# Autodesk Inventor assembly: foreArm
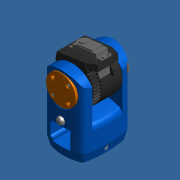
[picture p0: Inventor's stored thumbnail of the model, 180x180]
Saved by Autodesk Inventor 2014 SP2 (Build 180246200, 246)
## iProperties
Created: 2014-12-14
Part Number: foreArm
Document SubType Name: Assembly
Designer: 4ndreas
Mass: 1030.82 g
Surface Area: 1484.59 cm^2
Volume: 608.467 cm^3
Density: 1.69413 g/cm^3
Author: 4ndreas
## Documents named in this file (21)
- C:\Users\4ndreas\Documents\Inventor\RobotARm\foreArm.iam
- C:\Users\4ndreas\Documents\Inventor\RobotARm\RotaryArm.ipt
- C:\Users\4ndreas\Documents\Inventor\RobotARm\foreArm\Konstruktions-Assistent\Stirnräder1.iam
- C:\Users\4ndreas\Documents\Inventor\RobotARm\foreArm\Konstruktions-Assistent\Stirnräder2.iam
- C:\Users\4ndreas\Documents\Inventor\RobotARm\Nema11.ipt
- C:\Users\4ndreas\Documents\Inventor\RobotARm\foreArm\foreArm.ipt
- C:\Users\4ndreas\Documents\Inventor\RobotARm\foreArm\Konstruktions-Assistent\Stirnzahnrad12.ipt
- C:\Users\4ndreas\Documents\Inventor\Content Center Files\R2014\DIN 625 SKF - SKF 618_6_5mm.ipt
- C:\Users\4ndreas\Documents\Inventor\Content Center Files\R2014\de-DE\DIN BEARING(1)\DIN 625 SKF - SKF 626.ipt
- C:\Users\4ndreas\Documents\Inventor\RobotARm\Abdeckung.ipt
- C:\Users\4ndreas\Documents\Inventor\RobotARm\servo.ipt
- C:\Users\4ndreas\Documents\Inventor\Content Center Files\R2014\Leufter_30mm.ipt
- C:\Users\4ndreas\Documents\Inventor\RobotARm\foreArm\Konstruktions-Assistent\Welle1.iam
- C:\Users\4ndreas\Documents\Inventor\RobotARm\6mm Wellen klemme.ipt
- C:\Users\4ndreas\Documents\Inventor\Content Center Files\R2014\de-DE\DIN 913\DIN 913 - M3 x 4.ipt
- C:\Users\4ndreas\Documents\Inventor\Content Center Files\R2014\de-DE\DIN 931-1\DIN 931-1 - M6 x 35.ipt
- C:\Users\4ndreas\Documents\Inventor\Content Center Files\R2014\de-DE\DIN 433-1  A\DIN 433 - 6,4.ipt
- C:\Users\4ndreas\Documents\Inventor\Content Center Files\R2014\de-DE\DIN 985\DIN 985 - M6.ipt
- C:\Users\4ndreas\Documents\Inventor\Content Center Files\R2014\de-DE\DIN 912\DIN 912 - M4 x 0,7 x 25 x 23,25.ipt
- C:\Users\4ndreas\Documents\Inventor\Content Center Files\R2014\de-DE\DIN 934\DIN 934 - M4 x 0,7.ipt
- C:\Users\4ndreas\Documents\Inventor\Content Center Files\R2014\de-DE\DIN EN ISO 7046-2 H\DIN EN ISO 7046-2 H - M3x10 - 8.8 - H1.ipt
## Components (30 placed, 19 different names)
1. RotaryArm:1 — Passend:3, Passend:5, Passend:7, Passend:10, Winkel:1, Fluchtend:1, Passend:15, Passend:17, Passend:22, Passend:23, Passend:24, Passend:25, Passend:26, Passend:27, Passend:28, Fluchtend:2, Passend:29, Passend:30, Winkel:2, Winkel:3, Passend:38, Passend:39, Passend:40, Passend:41, Passend:42, Passend:43, Winkel:4, Fluchtend:4, Passend:53, Passend:54, Passend:59, Passend:60, Fluchtend:5, Passend:64, Passend:65, Winkel:6, Winkel:7, Passend:68, Passend:69, Passend:70
2. Stirnräder:1 [sub-assembly] — Passend:1, Passend:2, Passend:10, Fluchtend:3
3. Stirnräder:2 [sub-assembly] — Passend:13, Passend:14, Passend:15, Passend:16
4. Nema11:1 — Passend:11, Winkel:1, Passend:41
5. foreArm:1 — Passend:17, Passend:18, Drehung:1, Passend:36, Passend:37, Passend:57, Passend:58
6. Stirnzahnrad1:1 — Passend:19, Passend:20, Drehung:1
7. DIN 625 SKF 618/6:1 — Passend:21, Passend:24, Passend:46
8. DIN 625 SKF 618/6:2 — Passend:22, Passend:23
9. DIN 625 SKF 626:1 — Passend:26, Passend:27, Passend:49, Passend:50
10. DIN 625 SKF 626:2 — Passend:25, Passend:28, Passend:47, Passend:48
11. Abdeckung:1 — Passend:29, Passend:30, Passend:31, Passend:32, Passend:66, Passend:67
12. servo:1 — Passend:35, Passend:37, Winkel:3
13. Abdeckung:2 — Passend:38, Passend:39, Passend:40
14. Leufter_30mm:1 — Passend:42, Passend:43, Winkel:4
15. Welle:1 [sub-assembly] — Passend:44, Fluchtend:3, Passend:45
16. 6mm Wellen klemme:1 — Fluchtend:4, Passend:45, Passend:46, Zylindrisch:1
17. DIN 913 M3 x 4:1 — Zylindrisch:1
18. DIN 931-1 - ersetzt durch DIN EN 24014 M6 x 35:1 — Passend:47, Passend:48, Passend:52, Passend:56
19. DIN 931-1 - ersetzt durch DIN EN 24014 M6 x 35:2 — Passend:49, Passend:50, Passend:51, Passend:55
20. DIN 433-1 A 6,4:1 — Passend:51, Passend:53
21. DIN 433-1 A 6,4:2 — Passend:52, Passend:54
22. DIN 985 - ersetzt durch DIN EN ISO 10511 M6:1 — Passend:56, Passend:57, Winkel:5
23. DIN 985 - ersetzt durch DIN EN ISO 10511 M6:2 — Passend:55, Passend:58, Winkel:5
24. DIN 912 - ersetzt durch DIN EN ISO 4762 M4 x 25:2 — Passend:59, Fluchtend:5, Passend:61, Passend:62
25. DIN 912 - ersetzt durch DIN EN ISO 4762 M4 x 25:1 — Passend:60, Passend:61, Passend:63
26. DIN 934 - ersetzt durch DIN EN 24032/28673/28674 M4:1 — Passend:63, Passend:65, Winkel:6
27. DIN 934 - ersetzt durch DIN EN 24032/28673/28674 M4:2 — Passend:62, Passend:64, Winkel:7
28. DIN EN ISO 7046-2 H M3x10 - 8.8 - H1:1 — Passend:67, Fluchtend:6
29. DIN EN ISO 7046-2 H M3x10 - 8.8 - H1:2 — Passend:66, Fluchtend:6
30. Abdeckung:3 — Passend:68, Passend:69, Passend:70
## Relationships (82: Mate 67, Angle 7, Flush 6, RelateRotation 1, CylindricalJoint 1)
- Passend:1 [Mate]: Stirnräder:1
- Passend:2 [Mate]: Stirnräder:1
- Passend:3 [Mate]: RotaryArm:1
- Passend:4 [Mate]
- Passend:5 [Mate]: RotaryArm:1
- Passend:6 [Mate]
- Passend:7 [Mate]: RotaryArm:1
- Passend:10 [Mate]: RotaryArm:1 ↔ Stirnräder:1
- Passend:11 [Mate]: Nema11:1
- Winkel:1 [Angle] (0 deg): RotaryArm:1 ↔ Nema11:1
- Fluchtend:1 [Flush] (2 mm): RotaryArm:1
- Passend:13 [Mate]: Stirnräder:2
- Passend:14 [Mate]: Stirnräder:2
- Passend:15 [Mate]: RotaryArm:1 ↔ Stirnräder:2
- Passend:16 [Mate]: Stirnräder:2
- Passend:17 [Mate]: RotaryArm:1 ↔ foreArm:1
- Passend:18 [Mate]: foreArm:1
- Passend:19 [Mate]: Stirnzahnrad1:1
- Passend:20 [Mate]: Stirnzahnrad1:1
- Drehung:1 [RelateRotation] (0.3333 ul): foreArm:1 ↔ Stirnzahnrad1:1
- Passend:21 [Mate]: DIN 625 SKF 618/6:1
- Passend:22 [Mate]: RotaryArm:1 ↔ DIN 625 SKF 618/6:2
- Passend:23 [Mate]: RotaryArm:1 ↔ DIN 625 SKF 618/6:2
- Passend:24 [Mate]: RotaryArm:1 ↔ DIN 625 SKF 618/6:1
- Passend:25 [Mate]: RotaryArm:1 ↔ DIN 625 SKF 626:2
- Passend:26 [Mate]: RotaryArm:1 ↔ DIN 625 SKF 626:1
- Passend:27 [Mate]: RotaryArm:1 ↔ DIN 625 SKF 626:1
- Passend:28 [Mate]: RotaryArm:1 ↔ DIN 625 SKF 626:2
- Fluchtend:2 [Flush] (2 mm): RotaryArm:1
- Passend:29 [Mate]: RotaryArm:1 ↔ Abdeckung:1
- Passend:30 [Mate] (-4 mm): RotaryArm:1 ↔ Abdeckung:1
- Passend:31 [Mate]: Abdeckung:1
- Passend:32 [Mate]: Abdeckung:1
- Passend:33 [Mate]
- Passend:34 [Mate]
- Winkel:2 [Angle] (0 deg): RotaryArm:1
- Passend:35 [Mate]: servo:1
- Passend:36 [Mate]: foreArm:1
- Passend:37 [Mate]: foreArm:1 ↔ servo:1
- Winkel:3 [Angle] (0 deg): RotaryArm:1 ↔ servo:1
- Passend:38 [Mate]: RotaryArm:1 ↔ Abdeckung:2
- Passend:39 [Mate]: RotaryArm:1 ↔ Abdeckung:2
- Passend:40 [Mate]: RotaryArm:1 ↔ Abdeckung:2
- Passend:41 [Mate]: RotaryArm:1 ↔ Nema11:1
- Passend:42 [Mate]: RotaryArm:1 ↔ Leufter_30mm:1
- Passend:43 [Mate]: RotaryArm:1 ↔ Leufter_30mm:1
- Winkel:4 [Angle] (0 deg): RotaryArm:1 ↔ Leufter_30mm:1
- Passend:44 [Mate]: Welle:1
- Fluchtend:3 [Flush] (8 mm): Stirnräder:1 ↔ Welle:1
- Fluchtend:4 [Flush] (-9.5 mm): RotaryArm:1 ↔ 6mm Wellen klemme:1
- Passend:45 [Mate]: Welle:1 ↔ 6mm Wellen klemme:1
- Passend:46 [Mate]: DIN 625 SKF 618/6:1 ↔ 6mm Wellen klemme:1
- Zylindrisch:1 [CylindricalJoint]: 6mm Wellen klemme:1 ↔ DIN 913 M3 x 4:1
- Passend:47 [Mate]: DIN 625 SKF 626:2 ↔ DIN 931-1 - ersetzt durch DIN EN 24014 M6 x 35:1
- Passend:48 [Mate]: DIN 625 SKF 626:2 ↔ DIN 931-1 - ersetzt durch DIN EN 24014 M6 x 35:1
- Passend:49 [Mate]: DIN 625 SKF 626:1 ↔ DIN 931-1 - ersetzt durch DIN EN 24014 M6 x 35:2
- Passend:50 [Mate]: DIN 625 SKF 626:1 ↔ DIN 931-1 - ersetzt durch DIN EN 24014 M6 x 35:2
- Passend:51 [Mate]: DIN 931-1 - ersetzt durch DIN EN 24014 M6 x 35:2 ↔ DIN 433-1 A 6,4:1
- Passend:52 [Mate]: DIN 931-1 - ersetzt durch DIN EN 24014 M6 x 35:1 ↔ DIN 433-1 A 6,4:2
- Passend:53 [Mate]: RotaryArm:1 ↔ DIN 433-1 A 6,4:1
- Passend:54 [Mate]: RotaryArm:1 ↔ DIN 433-1 A 6,4:2
- Passend:55 [Mate]: DIN 931-1 - ersetzt durch DIN EN 24014 M6 x 35:2 ↔ DIN 985 - ersetzt durch DIN EN ISO 10511 M6:2
- Passend:56 [Mate]: DIN 931-1 - ersetzt durch DIN EN 24014 M6 x 35:1 ↔ DIN 985 - ersetzt durch DIN EN ISO 10511 M6:1
- Passend:57 [Mate]: foreArm:1 ↔ DIN 985 - ersetzt durch DIN EN ISO 10511 M6:1
- Passend:58 [Mate]: foreArm:1 ↔ DIN 985 - ersetzt durch DIN EN ISO 10511 M6:2
- Winkel:5 [Angle] (0 deg): DIN 985 - ersetzt durch DIN EN ISO 10511 M6:1 ↔ DIN 985 - ersetzt durch DIN EN ISO 10511 M6:2
- Passend:59 [Mate]: RotaryArm:1 ↔ DIN 912 - ersetzt durch DIN EN ISO 4762 M4 x 25:2
- Passend:60 [Mate]: RotaryArm:1 ↔ DIN 912 - ersetzt durch DIN EN ISO 4762 M4 x 25:1
- Fluchtend:5 [Flush]: RotaryArm:1 ↔ DIN 912 - ersetzt durch DIN EN ISO 4762 M4 x 25:2
- Passend:61 [Mate] (5.5 mm): DIN 912 - ersetzt durch DIN EN ISO 4762 M4 x 25:2 ↔ DIN 912 - ersetzt durch DIN EN ISO 4762 M4 x 25:1
- Passend:62 [Mate]: DIN 912 - ersetzt durch DIN EN ISO 4762 M4 x 25:2 ↔ DIN 934 - ersetzt durch DIN EN 24032/28673/28674 M4:2
- Passend:63 [Mate]: DIN 912 - ersetzt durch DIN EN ISO 4762 M4 x 25:1 ↔ DIN 934 - ersetzt durch DIN EN 24032/28673/28674 M4:1
- Passend:64 [Mate]: RotaryArm:1 ↔ DIN 934 - ersetzt durch DIN EN 24032/28673/28674 M4:2
- Passend:65 [Mate]: RotaryArm:1 ↔ DIN 934 - ersetzt durch DIN EN 24032/28673/28674 M4:1
- Winkel:6 [Angle] (0 deg): RotaryArm:1 ↔ DIN 934 - ersetzt durch DIN EN 24032/28673/28674 M4:1
- Winkel:7 [Angle] (0 deg): RotaryArm:1 ↔ DIN 934 - ersetzt durch DIN EN 24032/28673/28674 M4:2
- Passend:66 [Mate]: Abdeckung:1 ↔ DIN EN ISO 7046-2 H M3x10 - 8.8 - H1:2
- Passend:67 [Mate]: Abdeckung:1 ↔ DIN EN ISO 7046-2 H M3x10 - 8.8 - H1:1
- Fluchtend:6 [Flush]: DIN EN ISO 7046-2 H M3x10 - 8.8 - H1:1 ↔ DIN EN ISO 7046-2 H M3x10 - 8.8 - H1:2
- Passend:68 [Mate]: RotaryArm:1 ↔ Abdeckung:3
- Passend:69 [Mate]: RotaryArm:1 ↔ Abdeckung:3
- Passend:70 [Mate]: RotaryArm:1 ↔ Abdeckung:3
